# Autodesk Inventor assembly: ASY MSC 800.1 gills base
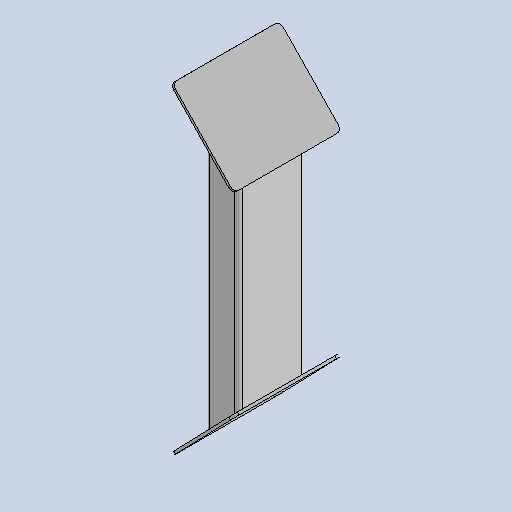
[picture p0: Inventor's stored thumbnail of the model, 512x512]
Saved by Autodesk Inventor 2025 (Build 290162010, 162A)
## iProperties
Created: 2024-09-02
Part Number: ASY MSC 800.1 gills base
Document SubType Name: Assembly
Designer: admin
Mass: 2289.28 g
Surface Area: 1980.66 cm^2
Volume: 290.028 cm^3
Density: 7.8933 g/cm^3
Stock Number: ASY МОО 800.1 основание жабр
Author: admin
## Documents named in this file (3)
- C:\Users\pokla\Documents\Inventor\Отстойник осветлитель\Manturovo_Se-clar-Gleb\ASY MSC 089 gills base.iam
- C:\Users\pokla\Documents\Inventor\Отстойник осветлитель\Manturovo_Se-clar-Gleb\MSC 085 bottom support gills.ipt
- C:\Users\pokla\Documents\Inventor\Отстойник осветлитель\Manturovo_Se-clar-Gleb\MSC 087 bottom plate gills.ipt
## Components (3 placed, 2 different names)
1. MSC 085 bottom support gills:1
2. MSC 087 bottom plate gills:2
3. MSC 087 bottom plate gills:1
## Relationships (2: WeldJoint 2)
- [WeldJoint]: MSC 085 bottom support gills:1 ↔ MSC 087 bottom plate gills:1
- [WeldJoint]: MSC 085 bottom support gills:1 ↔ MSC 087 bottom plate gills:2
